# Autodesk Inventor assembly: KickerUnit
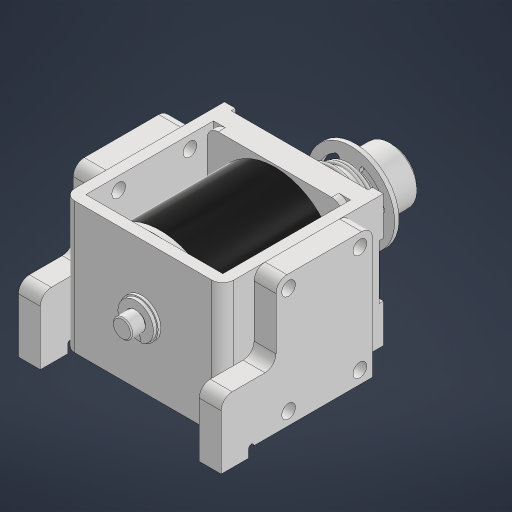
[picture p0: Inventor's stored thumbnail of the model, 512x512]
Saved by Autodesk Inventor 2024.2 (Build 282272000, 272)
## iProperties
Created: 2023-12-22
Part Number: KickerUnit
Document SubType Name: Assembly
Designer: Hanaoka
Author: Hanaoka
## Documents named in this file (4)
- G:\共有ドライブ\reRo\05_個人\hanaoka\inventor\KickerUnit.iam
- G:\共有ドライブ\reRo\05_個人\hanaoka\inventor\cb1029\cb1029.iam
- G:\共有ドライブ\reRo\05_個人\hanaoka\inventor\SolenoidMount.ipt
- G:\共有ドライブ\reRo\05_個人\hanaoka\inventor\SolenoidMount_MIR.ipt
## Components (3 placed, 3 different names)
1. cb1029:1 [sub-assembly] — メイト:1, フラッシュ:1, 正接:1, フラッシュ:2, フラッシュ:3
2. SolenoidMount:1 — フラッシュ:2, フラッシュ:3
3. SolenoidMount_MIR:1
## Relationships (5: Flush 3, Mate 1, Tangent 1)
- メイト:1 [Mate]: cb1029:1
- フラッシュ:1 [Flush]: cb1029:1
- 正接:1 [Tangent] (-1.75 mm): cb1029:1
- フラッシュ:2 [Flush]: cb1029:1 ↔ SolenoidMount:1
- フラッシュ:3 [Flush]: cb1029:1 ↔ SolenoidMount:1
